# Autodesk Inventor assembly: СБ_Корпус
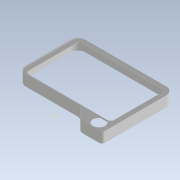
[picture p0: Inventor's stored thumbnail of the model, 180x180]
Saved by Autodesk Inventor 2021.2 (Build 252289000, 289)
## iProperties
Created: 2022-12-06
Part Number: СБ_Корпус
Document SubType Name: Assembly
Designer: Королев В. В.
Mass: 158.294 g
Surface Area: 1670.49 cm^2
Volume: 154.849 cm^3
Density: 1.02224 g/cm^3
Author: Королев В. В.
## Documents named in this file (4)
- C:\Users\Voodoo\Documents\Inventor\АБТ_Инфотабло\СБ_Корпус.iam
- C:\Users\Voodoo\Documents\Inventor\АБТ_Инфотабло\Обечайка часть 1.ipt
- C:\Users\Voodoo\Documents\Inventor\АБТ_Инфотабло\Обечайка часть 2.ipt
- C:\Users\Voodoo\Documents\Inventor\АБТ_Инфотабло\СБ_Лицевой лист.iam
## Components (3 placed, 3 different names)
1. Обечайка часть 1:1
2. Обечайка часть 2:1
3. СБ_Лицевой лист:1 [sub-assembly]
## Relationships (6: Flush 3, Mate 3)
- [Flush]: Обечайка часть 1:1 ↔ Обечайка часть 2:1
- [Mate]: Обечайка часть 1:1 ↔ Обечайка часть 2:1
- [Flush]: Обечайка часть 1:1 ↔ Обечайка часть 2:1
- [Flush] (2 mm): Обечайка часть 2:1 ↔ СБ_Лицевой лист:1
- [Mate]: Обечайка часть 1:1 ↔ СБ_Лицевой лист:1
- [Mate]: Обечайка часть 2:1 ↔ СБ_Лицевой лист:1
